# Autodesk Inventor assembly: ABD_Slider_Set
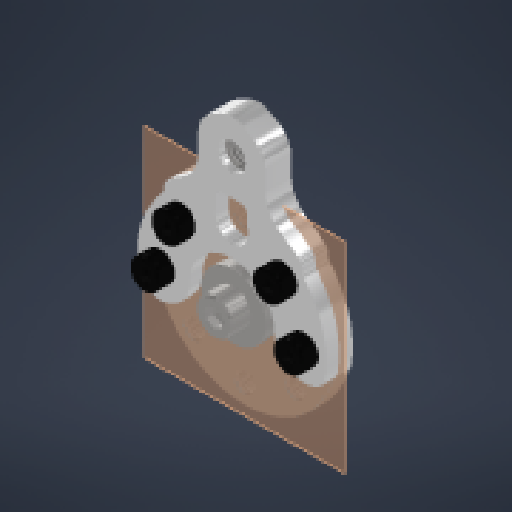
[picture p0: Inventor's stored thumbnail of the model, 512x512]
Saved by Autodesk Inventor 2024.3 (Build 283343000, 343)
## iProperties
Created: 2024-02-15
Part Number: ABD_Slider_Set
Document SubType Name: Assembly
Designer: ASUS
Author: ASUS
## Documents named in this file (6)
- C:\Users\ASUS\Desktop\test\v3_Frame\ABD_Slider_Set_v3.iam
- C:\Users\ASUS\Desktop\test\ROBOTIS(Inventor 2024 ver.)\HORN\64-106Horn.ipt
- C:\Users\ASUS\Desktop\test\v3_Frame\MISUMI\CSH-STN-M3-10.ipt
- C:\Users\ASUS\Desktop\test\v3_Frame\Slider_crank_horn_v3.ipt
- C:\Users\ASUS\Documents\Inventor\Content Center Files\R2024\ko-KR\ANSI B 18.2.4.1 M(1)\ANSI B 18.2.4.1 M - M4 x 0.7Style 1.ipt
- C:\Users\ASUS\Desktop\test\v3_Frame\MISUMI\CSH-ST-M2_5-4.ipt
## Components (8 placed, 5 different names)
1. 64-106Horn:1 — 삽입:3, 삽입:4
2. CSH-STN-M3-10:1 — 삽입:3
3. 6각 너트 미터 M4 x 0.7:1 — 각도:1, 각도:2, 삽입:5
4. Slider_crank_horn_v3:1 — 삽입:4, 각도:2, 삽입:5, 삽입:6, 삽입:7, 삽입:8, 삽입:9
5. CSH-ST-M2_5-4:1 — 삽입:9
6. CSH-ST-M2_5-4:2 — 삽입:6
7. CSH-ST-M2_5-4:3 — 삽입:7
8. CSH-ST-M2_5-4:4 — 삽입:8
## Relationships (9: Insert 7, Angle 2)
- 삽입:3 [Insert]: 64-106Horn:1 ↔ CSH-STN-M3-10:1
- 각도:1 [Angle] (0 deg): 6각 너트 미터 M4 x 0.7:1
- 삽입:4 [Insert]: 64-106Horn:1 ↔ Slider_crank_horn_v3:1
- 각도:2 [Angle] (0 deg): 6각 너트 미터 M4 x 0.7:1 ↔ Slider_crank_horn_v3:1
- 삽입:5 [Insert]: 6각 너트 미터 M4 x 0.7:1 ↔ Slider_crank_horn_v3:1
- 삽입:6 [Insert]: Slider_crank_horn_v3:1 ↔ CSH-ST-M2_5-4:2
- 삽입:7 [Insert]: Slider_crank_horn_v3:1 ↔ CSH-ST-M2_5-4:3
- 삽입:8 [Insert]: Slider_crank_horn_v3:1 ↔ CSH-ST-M2_5-4:4
- 삽입:9 [Insert]: Slider_crank_horn_v3:1 ↔ CSH-ST-M2_5-4:1
